# Autodesk Inventor assembly: SerV2
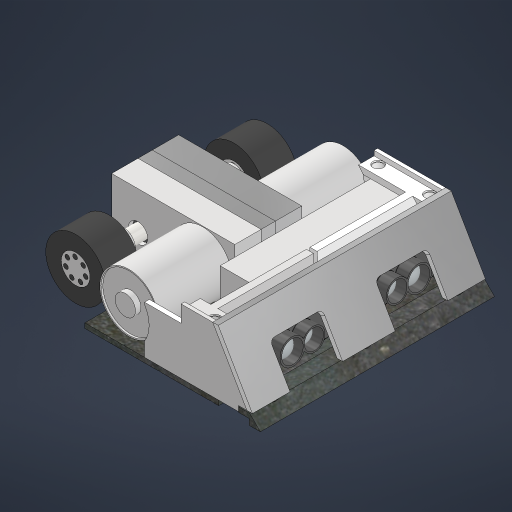
[picture p0: Inventor's stored thumbnail of the model, 512x512]
Saved by Autodesk Inventor 2023 (Build 270158000, 158)
## iProperties
Created: 2024-01-12
Part Number: SerV2
Document SubType Name: Assembly
Designer: Michał
Author: Michał
## Documents named in this file (11)
- D:\Projekty\Roboilo\Ser\3D\3D\V2\SerV2.iam
- D:\Projekty\Roboilo\Ser\3D\3D\V2\Blacha.ipt
- D:\Projekty\Roboilo\Ser\3D\3D\Plug2.ipt
- D:\Projekty\Roboilo\Ser\3D\3D\V2\bok.ipt
- D:\Projekty\Roboilo\Ser\3D\3D\V2\mini_Lidar.ipt
- D:\Projekty\Roboilo\Ser\3D\3D\V2\bok_MIR.ipt
- D:\Projekty\Roboilo\Ser\3D\3D\V2\mini_Lidar_MIR1.ipt
- D:\Projekty\Roboilo\Ser\3D\3D\V2\Naped.iam
- D:\Projekty\Roboilo\Ser\3D\3D\V2\Przod.ipt
- D:\Projekty\Roboilo\Ser\3D\3D\V2\akumulator.ipt
- D:\Projekty\Roboilo\Ser\3D\3D\V2\bok_MIR_MIR.ipt
## Components (10 placed, 10 different names)
1. Blacha:1 — Mate:1, Mate:2, Flush:1, Flush:2, Mate:8, Flush:4, Mate:9
2. Plug2:1 — Mate:1, Mate:2, Mate:12, Angle:1
3. bok:1 — Flush:1, Flush:2, Insert:3, Insert:4
4. mini_Lidar:1 — Insert:3, Insert:4
5. bok_MIR:1 — Insert:5, Insert:6, Mate:10, Mate:11
6. mini_Lidar_MIR1:1 — Insert:5, Insert:6
7. Naped:1 [sub-assembly] — Mate:8
8. Przod:1 — Flush:4
9. akumulator:1 — Mate:9, Mate:10, Mate:11
10. bok_MIR_MIR:1
## Relationships (15: Mate 7, Insert 4, Flush 3, Angle 1)
- Mate:1: Blacha:1 ↔ Plug2:1
- Mate:2: Blacha:1 ↔ Plug2:1
- Flush:1: Blacha:1 ↔ bok:1
- Flush:2: Blacha:1 ↔ bok:1
- Insert:3: bok:1 ↔ mini_Lidar:1
- Insert:4: bok:1 ↔ mini_Lidar:1
- Mate:8: Blacha:1 ↔ Naped:1
- Flush:4: Blacha:1 ↔ Przod:1
- Insert:5: bok_MIR:1 ↔ mini_Lidar_MIR1:1
- Insert:6: bok_MIR:1 ↔ mini_Lidar_MIR1:1
- Mate:9: Blacha:1 ↔ akumulator:1
- Mate:10 (0.1 mm): bok_MIR:1 ↔ akumulator:1
- Mate:11 (0.5 mm): bok_MIR:1 ↔ akumulator:1
- Mate:12: Plug2:1
- Angle:1 (0 deg): Plug2:1
